# Autodesk Inventor assembly: Driveshaft Plate Assembly
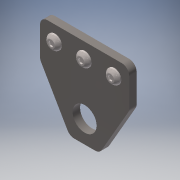
[picture p0: Inventor's stored thumbnail of the model, 180x180]
Saved by Autodesk Inventor 2017 (Build 210142000, 142)
## iProperties
Created: 2017-01-04
Part Number: Driveshaft Plate Assembly
Document SubType Name: Assembly
Designer: Ali
Author: Ali
## Documents named in this file (3)
- C:\Users\Ali\Desktop\roboticFarm-master\Models2\Gantry\Ali\Driveshaft Plate Assembly.iam
- C:\Users\Ali\Desktop\roboticFarm-master\Models2\Gantry\Ali\Driveshaft Plate.ipt
- C:\Users\Ali\Desktop\roboticFarm-master\Models2\Gantry\Ali\M5 Screw with Tee Nut.iam
## Components (4 placed, 2 different names)
1. Driveshaft Plate:1 — Rigid:1, Rigid:2, Rigid:3
2. M5 Screw with Tee Nut:1 [sub-assembly] — Rigid:3
3. M5 Screw with Tee Nut:3 [sub-assembly] — Rigid:1
4. M5 Screw with Tee Nut:4 [sub-assembly] — Rigid:2
## Relationships (3: WeldJoint 3)
- Rigid:1 [WeldJoint]: Driveshaft Plate:1 ↔ M5 Screw with Tee Nut:3
- Rigid:2 [WeldJoint]: Driveshaft Plate:1 ↔ M5 Screw with Tee Nut:4
- Rigid:3 [WeldJoint]: Driveshaft Plate:1 ↔ M5 Screw with Tee Nut:1
